# Autodesk Inventor assembly: Puzzle
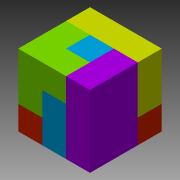
[picture p0: Inventor's stored thumbnail of the model, 180x180]
Saved by Autodesk Inventor 2015 (Build 190159000, 159)
## iProperties
Created: 2014-12-18
Part Number: Puzzle
Document SubType Name: Assembly
Designer: 1750019
Author: 1750019
## Documents named in this file (6)
- D:\RDrive\PLTW IED\PuzzleCube\Puzzle.iam
- D:\RDrive\PLTW IED\PuzzleCube\1.ipt
- D:\RDrive\PLTW IED\PuzzleCube\2.ipt
- D:\RDrive\PLTW IED\PuzzleCube\3.ipt
- D:\RDrive\PLTW IED\PuzzleCube\4.ipt
- D:\RDrive\PLTW IED\PuzzleCube\5.ipt
## Components (5 placed, 5 different names)
1. 1:1 — Flush:1, Flush:2, Mate:1, Flush:4, Mate:2, Flush:7, Flush:8
2. 2:1 — Mate:4, Flush:8, Flush:9, Flush:10
3. 3:1 — Flush:1, Flush:2, Mate:1, Flush:3, Flush:5, Mate:3, Flush:9, Flush:10
4. 4:1 — Flush:3, Flush:4, Flush:5, Flush:6, Mate:4
5. 5:1 — Mate:2, Flush:6, Mate:3, Flush:7
## Relationships (14: Flush 10, Mate 4)
- Flush:1: 1:1 ↔ 3:1
- Flush:2: 1:1 ↔ 3:1
- Mate:1: 1:1 ↔ 3:1
- Flush:3: 3:1 ↔ 4:1
- Flush:4: 1:1 ↔ 4:1
- Flush:5: 3:1 ↔ 4:1
- Mate:2: 1:1 ↔ 5:1
- Flush:6: 4:1 ↔ 5:1
- Mate:3: 3:1 ↔ 5:1
- Flush:7: 1:1 ↔ 5:1
- Mate:4: 2:1 ↔ 4:1
- Flush:8: 1:1 ↔ 2:1
- Flush:9: 2:1 ↔ 3:1
- Flush:10: 2:1 ↔ 3:1
